# Autodesk Inventor assembly: Motor con encaje2
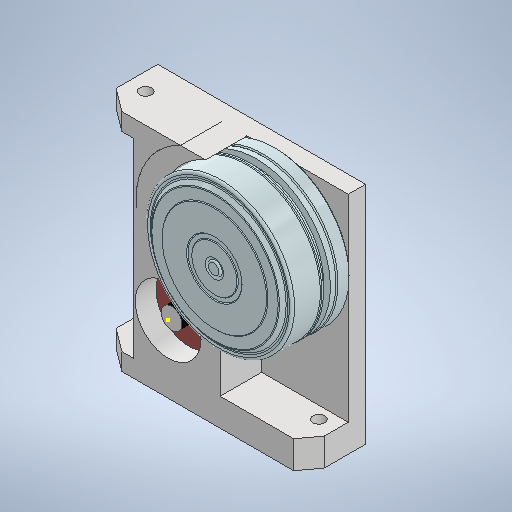
[picture p0: Inventor's stored thumbnail of the model, 512x512]
Saved by Autodesk Inventor 2025.1 (Build 291241000, 241)
## iProperties
Created: 2025-08-29
Part Number: Motor con encaje2
Document SubType Name: Assembly
Designer: paeze
Author: paeze
## Documents named in this file (5)
- C:\Users\paeze\Downloads\Base_Ruedas\28_08\Motor con encaje2.iam
- C:\Users\paeze\Downloads\Base_Ruedas\28_08\Mancal adaptado2.ipt
- C:\Users\paeze\Downloads\Base_Ruedas\28_08\Ruleman.ipt
- C:\Users\paeze\Downloads\Base_Ruedas\387266-ec45fl-30w-a-kabel\387266_ec45fl_30w_a_kabel\387266_ec45fl_30w_a_kabel\387266_ec45fl_30w_a_kabel.ipt
- C:\Users\paeze\Downloads\Base_Ruedas\Eje.ipt
## Components (4 placed, 4 different names)
1. Mancal adaptado2:1 — Rotational:1, Rigid:1
2. Ruleman:1 — Rotational:1, Rigid:2
3. 387266_ec45fl_30w_a_kabel:1 — Rigid:1
4. Eje:1 — Rigid:2
## Relationships (3: WeldJoint 2, RevoluteJoint 1)
- Rotational:1 [RevoluteJoint]: Mancal adaptado2:1 ↔ Ruleman:1
- Rigid:1 [WeldJoint] (-3 mm): Mancal adaptado2:1 ↔ 387266_ec45fl_30w_a_kabel:1
- Rigid:2 [WeldJoint] (5 mm): Ruleman:1 ↔ Eje:1
